# Autodesk Inventor assembly: 001_all
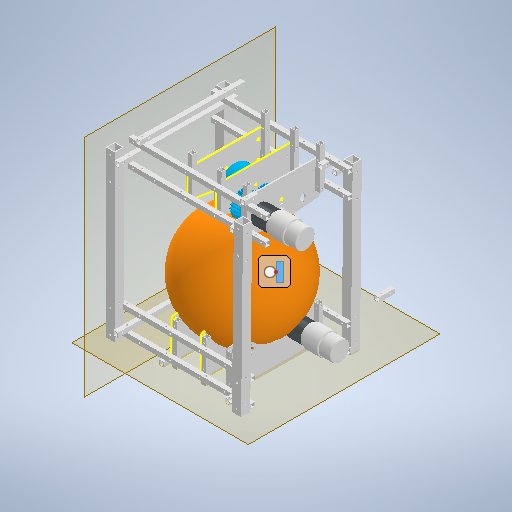
[picture p0: Inventor's stored thumbnail of the model, 512x512]
Saved by Autodesk Inventor 2025.1 (Build 291241000, 241)
## iProperties
Created: 2024-12-20
Part Number: 001_all
Document SubType Name: Assembly
Designer: yuki0520
Author: yuki0520
## Documents named in this file (7)
- C:\Users\yuki0520\OneDrive\ドキュメント\Inventor\2025_nhk\tanaka\nageru\smallring\001_all.iam
- C:\Users\yuki0520\OneDrive\ドキュメント\Inventor\2025_nhk\tanaka\nageru\smallring\001_ring.iam
- C:\Users\yuki0520\OneDrive\ドキュメント\Inventor\2025_nhk\tanaka\nageru\smallring\small_kaku_2020_tka.ipt
- C:\Users\yuki0520\OneDrive\ドキュメント\Inventor\2025_nhk\tanaka\object\ball.ipt
- C:\Users\yuki0520\OneDrive\ドキュメント\Inventor\2025_nhk\tanaka\nageru\smallring\small_kaku_1010_bridge_1020.ipt
- C:\Users\yuki0520\OneDrive\ドキュメント\Inventor\2025_nhk\tanaka\nageru\smallring\small_kaku_1010_santen_1020.ipt
- C:\Users\yuki0520\OneDrive\ドキュメント\Inventor\2025_nhk\tanaka\nageru\smallring\001_ring_shita.iam
## Components (13 placed, 6 different names)
1. 001_ring:1 [sub-assembly] — 挿入:48, 挿入:51, 挿入:52, 挿入:53, 挿入:55, 正接:3, 挿入:76
2. small_kaku_2020_tka:1 — 挿入:38, 挿入:46, 挿入:80
3. small_kaku_2020_tka:2 — 挿入:23, 挿入:43, メイト:3
4. small_kaku_2020_tka:3 — 挿入:39, 挿入:48, 挿入:50, 挿入:51, 挿入:77, 挿入:78
5. small_kaku_2020_tka:4 — 挿入:29, メイト:2, 挿入:52, 挿入:54, 挿入:55, 挿入:79
6. ball:1 — 正接:3
7. small_kaku_1010_bridge_1020:1 — 挿入:23, 挿入:29, 挿入:43, 挿入:53, 挿入:54
8. small_kaku_1010_bridge_1020:2 — 挿入:74
9. small_kaku_1010_santen_1020:1
10. small_kaku_1010_santen_1020:2 — 挿入:38, 挿入:46
11. small_kaku_1010_santen_1020:3 — 挿入:39, 挿入:50, 挿入:76
12. small_kaku_1010_santen_1020:4 — 挿入:73
13. 001_ring_shita:1 [sub-assembly] — 挿入:73, 挿入:74, 挿入:77, 挿入:78, 挿入:79, 挿入:80
## Relationships (23: Insert 20, Mate 2, Tangent 1)
- 挿入:23 [Insert]: small_kaku_2020_tka:2 ↔ small_kaku_1010_bridge_1020:1
- 挿入:29 [Insert]: small_kaku_2020_tka:4 ↔ small_kaku_1010_bridge_1020:1
- メイト:2 [Mate]: small_kaku_2020_tka:4
- 挿入:38 [Insert]: small_kaku_2020_tka:1 ↔ small_kaku_1010_santen_1020:2
- 挿入:39 [Insert]: small_kaku_2020_tka:3 ↔ small_kaku_1010_santen_1020:3
- 挿入:43 [Insert]: small_kaku_2020_tka:2 ↔ small_kaku_1010_bridge_1020:1
- 挿入:46 [Insert]: small_kaku_2020_tka:1 ↔ small_kaku_1010_santen_1020:2
- 挿入:48 [Insert]: 001_ring:1 ↔ small_kaku_2020_tka:3
- 挿入:50 [Insert]: small_kaku_2020_tka:3 ↔ small_kaku_1010_santen_1020:3
- 挿入:51 [Insert]: 001_ring:1 ↔ small_kaku_2020_tka:3
- 挿入:52 [Insert]: 001_ring:1 ↔ small_kaku_2020_tka:4
- 挿入:53 [Insert]: 001_ring:1 ↔ small_kaku_1010_bridge_1020:1
- 挿入:54 [Insert]: small_kaku_2020_tka:4 ↔ small_kaku_1010_bridge_1020:1
- 挿入:55 [Insert]: 001_ring:1 ↔ small_kaku_2020_tka:4
- 正接:3 [Tangent]: 001_ring:1 ↔ ball:1
- 挿入:73 [Insert]: small_kaku_1010_santen_1020:4 ↔ 001_ring_shita:1
- 挿入:74 [Insert]: small_kaku_1010_bridge_1020:2 ↔ 001_ring_shita:1
- 挿入:76 [Insert]: 001_ring:1 ↔ small_kaku_1010_santen_1020:3
- 挿入:77 [Insert]: small_kaku_2020_tka:3 ↔ 001_ring_shita:1
- 挿入:78 [Insert]: small_kaku_2020_tka:3 ↔ 001_ring_shita:1
- 挿入:79 [Insert]: small_kaku_2020_tka:4 ↔ 001_ring_shita:1
- 挿入:80 [Insert]: small_kaku_2020_tka:1 ↔ 001_ring_shita:1
- メイト:3 [Mate]: small_kaku_2020_tka:2
